# Autodesk Inventor assembly: Fixture Assembly
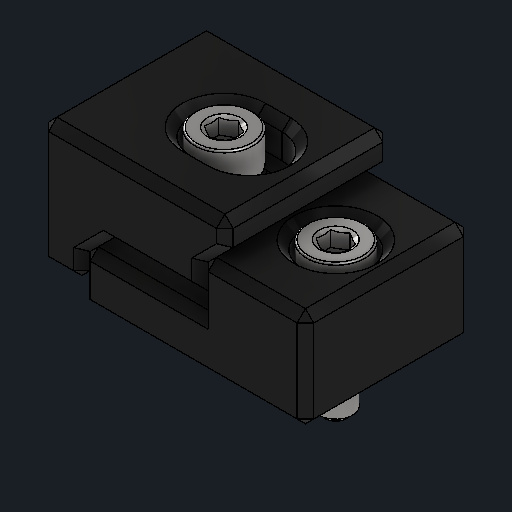
[picture p0: Inventor's stored thumbnail of the model, 512x512]
Saved by Autodesk Inventor 2026.2 (Build 302298000, 298)
## iProperties
Created: 2026-07-19
Part Number: Fixture Assembly
Document SubType Name: Assembly
Designer: JoshuaEah
Author: JoshuaEah
## Documents named in this file (5)
- C:\Users\JoshuaEah\Documents\GitHub\Designed-Trinkets\Guitar\Modular Pedalboard\Fixtures\M4 Version\Fixture Assembly (M4).iam
- C:\Users\JoshuaEah\Documents\GitHub\Designed-Trinkets\Guitar\Modular Pedalboard\Fixtures\M4 Version\Moving Jaw (M4).ipt
- C:\Users\JoshuaEah\Documents\GitHub\Designed-Trinkets\Guitar\Modular Pedalboard\Fixtures\M4 Version\Fixed Jaw (M4).ipt
- C:\Users\JoshuaEah\Documents\GitHub\Designed-Trinkets\Guitar\Modular Pedalboard\Hardware\M4x0.7 Hex Nut.ipt
- C:\Users\JoshuaEah\Documents\GitHub\Designed-Trinkets\Guitar\Modular Pedalboard\Hardware\M4x0.7x14mm SHCS.ipt
## Components (5 placed, 4 different names)
1. Fixed Jaw (M4):1 — Insert:1, Angle:2, Slider:1, Mate:2, Insert:2
2. Moving Jaw (M4):1 — Slider:1, Mate:1
3. M4x0.7 Hex Nut:1 — Insert:1, Angle:2
4. M4x0.7x14mm SHCS:1 — Mate:1, Mate:2
5. M4x0.7x14mm SHCS:2 — Insert:2
## Relationships (6: Insert 2, Mate 2, Angle 1, TranslationJoint 1)
- Insert:1: Fixed Jaw (M4):1 ↔ M4x0.7 Hex Nut:1
- Angle:2 (0 deg): Fixed Jaw (M4):1 ↔ M4x0.7 Hex Nut:1
- Slider:1 [TranslationJoint]: Fixed Jaw (M4):1 ↔ Moving Jaw (M4):1
- Mate:1: Moving Jaw (M4):1 ↔ M4x0.7x14mm SHCS:1
- Mate:2: Fixed Jaw (M4):1 ↔ M4x0.7x14mm SHCS:1
- Insert:2: Fixed Jaw (M4):1 ↔ M4x0.7x14mm SHCS:2
## Named parameters: travelDistance = 2.82843 mm, chamferSize = 1 mm, jawTravel = 3 mm
